# Autodesk Inventor assembly: frame
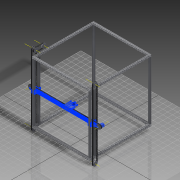
[picture p0: Inventor's stored thumbnail of the model, 180x180]
Saved by Autodesk Inventor 2013 (Build 170138000, 138)
## iProperties
Created: 2013-09-09
Part Number: frame
Document SubType Name: Assembly
Designer: Ian
Mass: 20029.5 g
Surface Area: 72396 cm^2
Volume: 16186.8 cm^3
Density: 1.2374 g/cm^3
Author: Ian
## Documents named in this file (6)
- C:\Users\Ian\Documents\Inventor\xyPartStorage\frame.iam
- C:\Users\Ian\Documents\Inventor\xyPartStorage\frame\Design Accelerator\Synchronous Belts Transmission1.iam
- C:\Users\Ian\Documents\Inventor\xyPartStorage\loader\xyArmature.iam
- C:\Users\Ian\Documents\Inventor\xyPartStorage\loader\sub-frame.iam
- C:\Users\Ian\Documents\Inventor\xyPartStorage\frame\Design Accelerator\Synchronous Belts Transmission2.iam
- C:\Users\Ian\Documents\Inventor\xyPartStorage\frame\Design Accelerator\Synchronous Belts Transmission3.iam
## Components (6 placed, 3 different names)
1. sub-frame:1 [sub-assembly] — Mate:55, Angle:1
2. Synchronous Belts Transmission:1 [sub-assembly] — Flush:1, Flush:3
3. xyArmature:1 [sub-assembly] — Flush:1, Flush:2, Mate:58
4. Synchronous Belts Transmission:2 [sub-assembly] — Flush:2, Mate:53, Mate:54, Mate:55, Mate:56, Mate:57, Mate:59, Mate:60
5. Synchronous Belts Transmission:3 [sub-assembly] — Mate:56, Mate:57, Mate:58
6. Synchronous Belts Transmission:4 [sub-assembly] — Mate:59, Mate:60, Mate:61, Mate:62
## Relationships (25: Mate 21, Flush 3, Angle 1)
- [Mate]: sub-frame:1 ↔ xyArmature:1
- [Mate]: sub-frame:1 ↔ xyArmature:1
- [Mate]: sub-frame:1 ↔ xyArmature:1
- [Mate]: sub-frame:1 ↔ xyArmature:1
- [Mate]: sub-frame:1 ↔ xyArmature:1
- [Mate]: sub-frame:1 ↔ xyArmature:1
- [Mate]: sub-frame:1 ↔ xyArmature:1
- [Mate]: sub-frame:1 ↔ xyArmature:1
- [Mate]: sub-frame:1 ↔ xyArmature:1
- [Mate]: Synchronous Belts Transmission:1 ↔ xyArmature:1
- [Mate] (-35.7124 mm): Synchronous Belts Transmission:1 ↔ xyArmature:1
- Flush:1 (7.62 mm): Synchronous Belts Transmission:1 ↔ xyArmature:1
- Flush:2 (12.7 mm): xyArmature:1 ↔ Synchronous Belts Transmission:2
- Flush:3 (-9.525 mm): Synchronous Belts Transmission:1
- Mate:53: Synchronous Belts Transmission:2
- Mate:54: Synchronous Belts Transmission:2
- Mate:55 (57.15 mm): sub-frame:1 ↔ Synchronous Belts Transmission:2
- Mate:56: Synchronous Belts Transmission:2 ↔ Synchronous Belts Transmission:3
- Mate:57: Synchronous Belts Transmission:2 ↔ Synchronous Belts Transmission:3
- Mate:58 (-12.7 mm): xyArmature:1 ↔ Synchronous Belts Transmission:3
- Mate:59: Synchronous Belts Transmission:2 ↔ Synchronous Belts Transmission:4
- Mate:60 (6.35 mm): Synchronous Belts Transmission:2 ↔ Synchronous Belts Transmission:4
- Mate:61: Synchronous Belts Transmission:4
- Angle:1 (0 deg): sub-frame:1
- Mate:62: Synchronous Belts Transmission:4
